# Autodesk Inventor assembly: Grundplatte_test
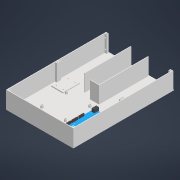
[picture p0: Inventor's stored thumbnail of the model, 180x180]
Saved by Autodesk Inventor 2021 (Build 250183000, 183)
## iProperties
Created: 2021-01-26
Part Number: Grundplatte_test
Document SubType Name: Assembly
Designer: Ctroi
Author: Ctroi
## Documents named in this file (5)
- G:\Roverprojekt\Github Projekt\Rover\Grundplatte_test.iam
- G:\Roverprojekt\Github Projekt\Rover\Grundplatte_hinten.ipt
- G:\Roverprojekt\Github Projekt\Rover\Grundplatte_vorne.ipt
- G:\Roverprojekt\Github Projekt\Rover\ArduinoMega.ipt
- G:\Roverprojekt\Github Projekt\Rover\Relais.ipt
## Components (4 placed, 4 different names)
1. Grundplatte_hinten:1 — Passend:1, Passend:2
2. Grundplatte_vorne:1 — Passend:1, Passend:2, Passend:3, Passend:4
3. ArduinoMega:1 — Passend:3, Passend:4
4. Relais:1
## Relationships (4: Mate 4)
- Passend:1 [Mate]: Grundplatte_hinten:1 ↔ Grundplatte_vorne:1
- Passend:2 [Mate]: Grundplatte_hinten:1 ↔ Grundplatte_vorne:1
- Passend:3 [Mate]: Grundplatte_vorne:1 ↔ ArduinoMega:1
- Passend:4 [Mate]: Grundplatte_vorne:1 ↔ ArduinoMega:1
